# Autodesk Inventor assembly: FTC Drivetrain V2
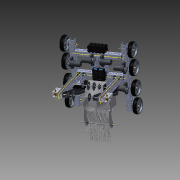
[picture p0: Inventor's stored thumbnail of the model, 180x180]
Saved by Autodesk Inventor 2015 (Build 190159000, 159)
## iProperties
Created: 2014-08-16
Part Number: FTC Drivetrain V2
Document SubType Name: Assembly
Designer: Vinay
Mass: 2195.41 g
Surface Area: 12375.9 cm^2
Volume: 2195.41 cm^3
Density: 1 g/cm^3
Author: Vinay
## Documents named in this file (38)
- C:\Working Folder\FTC Drivetrain V3.iam
- C:\Working Folder\CAD Models\Imported Components\Pitsco Education-739069\Pitsco Education-739069.ipt
- C:\Working Folder\CAD Models\FTC_Tetrix_KOP_Block_Party\Tetrix_Kit_FTC\Imported Components\tetrix_739089_2012\tetrix_739089_2012.ipt
- C:\Working Folder\CAD Models\FTC_Tetrix_KOP_Block_Party\Tetrix_Kit_FTC\Imported Components\tetrix_739083_motor_2012\tetrix_739083_motor_2012.ipt
- C:\Working Folder\CAD Models\Imported Components\Pitsco Education-739091\Pitsco Education-739091.ipt
- C:\Working Folder\CAD Models\Imported Components\Pitsco Education-739069\Pitsco Education-739069_MIR.ipt
- C:\Working Folder\CAD Models\FTC_Tetrix_KOP_Block_Party\Tetrix_Kit_FTC\Imported Components\tetrix_739089_2012\tetrix_739089_2012_MIR.ipt
- C:\Working Folder\CAD Models\FTC_Tetrix_KOP_Block_Party\Tetrix_Kit_FTC\Imported Components\tetrix_739083_motor_2012\tetrix_739083_motor_2012_MIR.ipt
- C:\Working Folder\CAD Models\Imported Components\Pitsco Education-739091\Pitsco Education-739091_MIR.ipt
- C:\Working Folder\CAD Models\FTC_Tetrix_KOP_Block_Party\Tetrix_Kit_FTC\Imported Components\tetrix_739062_2012\tetrix_739062_2012.ipt
- C:\Working Folder\CAD Models\Imported Components\Pitsco Education-739068\Pitsco Education-739068.ipt
- C:\Working Folder\CAD Models\FTC_Tetrix_KOP_Block_Party\Tetrix_Kit_FTC\Imported Components\tetrix_739088_2013\tetrix_739088_2013.ipt
- C:\Working Folder\CAD Models\FTC_Tetrix_KOP_Block_Party\Tetrix_Kit_FTC\Imported Components\tetrix_739079_2012\tetrix_739079_2012.iam
- C:\Working Folder\CAD Models\FTC_Tetrix_KOP_Block_Party\Tetrix_Kit_FTC\Imported Components\tetrix_739172_2012\tetrix_739172_2012.iam
- C:\Working Folder\CAD Models\Imported Components\Pitsco Education-739169\Pitsco Education-739169.ipt
- C:\Working Folder\CAD Models\FTC_Tetrix_KOP_Block_Party\Tetrix_Kit_FTC\Imported Components\tetrix_739165_sprk_25_16t_2013\tetrix_739165_sprk_25_16t_2013.ipt
- C:\Working Folder\CAD Models\FTC_Tetrix_KOP_Block_Party\Tetrix_Kit_FTC\Imported Components\tetrix_739092_2012\tetrix_739092_2012.iam
- C:\Working Folder\CAD Models\FTC_Tetrix_KOP_Block_Party\Tetrix_Kit_FTC\Imported Components\tetrix_739172_collar_2012\tetrix_739172_collar_2012.ipt
- C:\Working Folder\CAD Models\FTC_Tetrix_KOP_Block_Party\Tetrix_Kit_FTC\Imported Components\tetrix_739100_2012\tetrix_739100_2012.ipt
- C:\Working Folder\CAD Models\FTC_Tetrix_KOP_Block_Party\Tetrix_Kit_FTC\Imported Components\tetrix_739055_2012\tetrix_739055_2012.ipt
- C:\Working Folder\CAD Models\Imported Components\Pitsco Education-739066\Pitsco Education-739066.ipt
- C:\Working Folder\CAD Models\FTC_Tetrix_KOP_Block_Party\Tetrix_Kit_FTC\Imported Components\tetrix_739089_2012\tetrix_739089_2012_MIR1.ipt
- C:\Working Folder\CAD Models\FTC_Tetrix_KOP_Block_Party\Tetrix_Kit_FTC\Imported Components\tetrix_739083_motor_2012\tetrix_739083_motor_2012_MIR1.ipt
- C:\Working Folder\CAD Models\FTC_Tetrix_KOP_Block_Party\Tetrix_Kit_FTC\Imported Components\tetrix_739079_2012\tetrix_739079_2012_MIR.iam
- C:\Working Folder\CAD Models\FTC_Tetrix_KOP_Block_Party\Tetrix_Kit_FTC\Imported Components\tetrix_739165_sprk_25_16t_2013\tetrix_739165_sprk_25_16t_2013_MIR.ipt
- C:\Working Folder\CAD Models\Imported Components\Pitsco Education-739066\Pitsco Education-739066_MIR.ipt
- C:\Working Folder\CAD Models\FTC_Tetrix_KOP_Block_Party\Tetrix_Kit_FTC\Imported Components\tetrix_739089_2012\tetrix_739089_2012_MIR1_MIR.ipt
- C:\Working Folder\CAD Models\FTC_Tetrix_KOP_Block_Party\Tetrix_Kit_FTC\Imported Components\tetrix_739083_motor_2012\tetrix_739083_motor_2012_MIR1_MIR.ipt
- C:\Working Folder\CAD Models\FTC_Tetrix_KOP_Block_Party\Tetrix_Kit_FTC\Imported Components\tetrix_739079_2012\tetrix_739079_2012_MIR_MIR.iam
- C:\Working Folder\CAD Models\FTC_Tetrix_KOP_Block_Party\Tetrix_Kit_FTC\Imported Components\tetrix_739165_sprk_25_16t_2013\tetrix_739165_sprk_25_16t_2013_MIR_MIR.ipt
- C:\Working Folder\CAD Models\Long Axle 250mm.ipt
- C:\Working Folder\CAD Models\FTC_Tetrix_KOP_Block_Party\Tetrix_Kit_FTC\Imported Components\tetrix_739169_sprk_25_24t_2013\tetrix_739169_sprk_25_24t_2013.ipt
- C:\Working Folder\CAD Models\FTC_Tetrix_KOP_Block_Party\Tetrix_Kit_FTC\Imported Components\tetrix_739169_2012\tetrix_739169_2012.ipt
- C:\Working Folder\CAD Models\FTC_Tetrix_KOP_Block_Party\Tetrix_Kit_FTC\Imported Components\tetrix_739068_2012\tetrix_739068_2012.ipt
- C:\Working Folder\CAD Models\FTC_Tetrix_KOP_Block_Party\Tetrix_Kit_FTC\Imported Components\tetrix_991444_2012\tetrix_991444_2012.ipt
- C:\Working Folder\CAD Models\FTC_Tetrix_KOP_Block_Party\Tetrix_Kit_FTC\Imported Components\tetrix_739057_2012\tetrix_739057_2012.ipt
- C:\Working Folder\CAD Models\Imported Components\Pitsco Education-739375\Pitsco Education-739375.iam
- C:\Working Folder\CAD Models\GAME ELEMENT FINAL.iam
## Components (151 placed, 37 different names)
1. Pitsco Education-739069:1 — Mate:11, Mate:12, Mate:13, Mate:14, Mate:17, Mate:18, Mate:19, Mate:20, Mate:21, Mate:22, Mate:23, Mate:24, Mate:49, Mate:50, Mate:51, Mate:61, Mate:62, Mate:63, Mate:70, Mate:71, Mate:72, Mate:73, Flush:8, Flush:9, Flush:10, Flush:11, Mate:235, Mate:236, Mate:237, Mate:238, Mate:239, Mate:240, Mate:335, Flush:23
2. tetrix_739089_2012:1 — Mate:7, Flush:2, Mate:235, Mate:236, Mate:237
3. tetrix_739089_2012:2 — Mate:8, Flush:1, Mate:238, Mate:239, Mate:240
4. tetrix_739083_motor_2012:1 — Mate:7, Flush:2, Mate:86, Mate:87
5. tetrix_739083_motor_2012:2 — Mate:8, Flush:1, Mate:88, Mate:89
6. Pitsco Education-739091:1 — Mate:11, Mate:12, Mate:134, Mate:135
7. Pitsco Education-739091:3 — Mate:13, Mate:14, Mate:85, Mate:94
8. Pitsco Education-739091:4 — Mate:72, Mate:73, Mate:82, Mate:100
9. Pitsco Education-739091:5 — Mate:23, Mate:24, Mate:146, Mate:147
10. Pitsco Education-739091:6 — Mate:70, Mate:71, Mate:84, Mate:96
11. Pitsco Education-739091:7 — Mate:21, Mate:22, Mate:142, Mate:143
12. Pitsco Education-739091:10 — Mate:19, Mate:20, Mate:136, Mate:137
13. Pitsco Education-739091:11 — Mate:17, Mate:18, Mate:83, Mate:98
14. Pitsco Education-739069_MIR:1 — Mate:33, Mate:34, Mate:35, Mate:36, Mate:39, Mate:40, Mate:43, Mate:44, Mate:45, Mate:46, Mate:47, Mate:48, Mate:58, Mate:59, Mate:60, Mate:74, Mate:75, Mate:76, Mate:77, Flush:5, Flush:6, Mate:150, Flush:7, Mate:241, Mate:242, Mate:243, Mate:244, Mate:245, Mate:246
15. tetrix_739089_2012_MIR:1 — Flush:3, Mate:31, Mate:241, Mate:242, Mate:243
16. tetrix_739089_2012_MIR:2 — Flush:4, Mate:32, Mate:244, Mate:245, Mate:246
17. tetrix_739083_motor_2012_MIR:1 — Flush:3, Mate:31, Mate:90, Mate:91
18. tetrix_739083_motor_2012_MIR:2 — Flush:4, Mate:32, Mate:92, Mate:93
19. Pitsco Education-739091_MIR:1 — Mate:33, Mate:34, Mate:140, Mate:141
20. Pitsco Education-739091_MIR:2 — Mate:35, Mate:36, Mate:81, Mate:108
21. Pitsco Education-739091_MIR:3 — Mate:76, Mate:77, Mate:78, Mate:106
22. Pitsco Education-739091_MIR:4 — Mate:39, Mate:40, Mate:148, Mate:149
23. Pitsco Education-739091_MIR:5 — Mate:74, Mate:75, Mate:80, Mate:102
24. Pitsco Education-739091_MIR:6 — Mate:43, Mate:44, Mate:144, Mate:145
25. Pitsco Education-739091_MIR:7 — Mate:45, Mate:46, Mate:138, Mate:139
26. Pitsco Education-739091_MIR:8 — Mate:47, Mate:48, Mate:79, Mate:104
27. tetrix_739062_2012:2 — Mate:49, Mate:50, Mate:51, Mate:52, Mate:53, Mate:54
28. Pitsco Education-739068:1 — Mate:52, Mate:53, Mate:54, Mate:55, Mate:56, Mate:57, Mate:276, Mate:277, Flush:14, Flush:16, Mate:286, Mate:287, Mate:336
29. tetrix_739062_2012:5 — Mate:55, Mate:56, Mate:57, Mate:58, Mate:59, Mate:60
30. tetrix_739062_2012:6 — Mate:61, Mate:62, Mate:63, Mate:64, Mate:65, Mate:66, Mate:216
31. tetrix_739062_2012:7 — Mate:67, Mate:68, Mate:69
32. Pitsco Education-739068:2 — Mate:64, Mate:65, Mate:66, Mate:67, Mate:68, Mate:69, Mate:215, Mate:217, Mate:220, Mate:221, Mate:222, Mate:225, Mate:226, Mate:227, Mate:229, Mate:230, Mate:278, Mate:288, Mate:328, Mate:329
33. tetrix_739088_2013:1 — Mate:81, Mate:109, Flush:6, Mate:174, Mate:182, Mate:190
34. tetrix_739088_2013:2 — Mate:80, Mate:103, Flush:7, Mate:172, Mate:180, Mate:188, Mate:196
35. tetrix_739088_2013:3 — Mate:79, Mate:105, Mate:150, Mate:170, Mate:178, Mate:186, Mate:194
36. tetrix_739088_2013:4 — Mate:78, Mate:107, Flush:5, Mate:167, Mate:176, Mate:184
37. tetrix_739088_2013:5 — Mate:85, Mate:95, Flush:11, Mate:158, Mate:164, Mate:200
38. tetrix_739088_2013:6 — Mate:84, Mate:97, Flush:10, Mate:154, Mate:166, Mate:202
39. tetrix_739088_2013:7 — Mate:83, Mate:99, Flush:9, Mate:155, Mate:162, Mate:204
40. tetrix_739088_2013:8 — Mate:82, Mate:101, Flush:8, Mate:152, Mate:160, Mate:206
41. tetrix_739079_2012:1 [sub-assembly] — Mate:88, Mate:89, Mate:112, Mate:113
42. tetrix_739079_2012:2 [sub-assembly] — Mate:86, Mate:87, Mate:116, Mate:117
43. tetrix_739079_2012:3 [sub-assembly] — Mate:92, Mate:93, Mate:122, Mate:123
44. tetrix_739079_2012:4 [sub-assembly] — Mate:90, Mate:91, Mate:132, Mate:133
45. tetrix_739172_2012:1 [sub-assembly] — Mate:94, Mate:95, Mate:110, Mate:111
46. tetrix_739172_2012:2 [sub-assembly] — Mate:100, Mate:101, Mate:120, Mate:121
47. tetrix_739172_2012:3 [sub-assembly] — Mate:98, Mate:99, Mate:118, Mate:119
48. tetrix_739172_2012:4 [sub-assembly] — Mate:96, Mate:97, Mate:114, Mate:115
49. tetrix_739172_2012:6 [sub-assembly] — Mate:104, Mate:105, Mate:126, Mate:127
50. tetrix_739172_2012:7 [sub-assembly] — Mate:106, Mate:107, Mate:124, Mate:125
51. tetrix_739172_2012:8 [sub-assembly] — Mate:108, Mate:109, Mate:130, Mate:131
52. Pitsco Education-739169:1 — Mate:110, Mate:111, Mate:157
53. Pitsco Education-739169:2 — Mate:114, Mate:115, Mate:153
54. Pitsco Education-739169:3 — Mate:118, Mate:119, Mate:156
55. Pitsco Education-739169:4 — Mate:120, Mate:121, Mate:151
56. tetrix_739165_sprk_25_16t_2013:1 — Mate:122, Mate:123
57. tetrix_739165_sprk_25_16t_2013:2 — Mate:112, Mate:113
58. tetrix_739165_sprk_25_16t_2013:3 — Mate:116, Mate:117
59. Pitsco Education-739169:5 — Mate:124, Mate:125, Mate:168
60. Pitsco Education-739169:6 — Mate:126, Mate:127, Mate:169
61. Pitsco Education-739169:7 — Mate:130, Mate:131, Mate:173
62. Pitsco Education-739169:8 — Mate:128, Mate:129, Mate:171
63. tetrix_739165_sprk_25_16t_2013:4 — Mate:132, Mate:133
64. tetrix_739092_2012:1 [sub-assembly] — Mate:138, Mate:139
65. tetrix_739092_2012:2 [sub-assembly] — Mate:142, Mate:143
66. tetrix_739172_2012:5 [sub-assembly] — Mate:102, Mate:103, Mate:128, Mate:129
67. tetrix_739092_2012:3 [sub-assembly] — Mate:140, Mate:141
68. tetrix_739092_2012:4 [sub-assembly] — Mate:146, Mate:147
69. tetrix_739092_2012:5 [sub-assembly] — Mate:136, Mate:137
70. tetrix_739092_2012:6 [sub-assembly] — Mate:144, Mate:145
71. tetrix_739092_2012:7 [sub-assembly] — Mate:148, Mate:149
72. tetrix_739092_2012:8 [sub-assembly] — Mate:134, Mate:135
73. tetrix_739172_collar_2012:1 — Mate:163, Mate:164, Mate:199
74. tetrix_739172_collar_2012:2 — Mate:161, Mate:162, Mate:203
75. tetrix_739172_collar_2012:3 — Mate:159, Mate:160, Mate:205
76. tetrix_739172_collar_2012:4 — Mate:165, Mate:166, Mate:201
77. tetrix_739100_2012:1 — Mate:155, Mate:156, Mate:161
78. tetrix_739100_2012:2 — Mate:151, Mate:152, Mate:159
79. tetrix_739100_2012:3 — Mate:153, Mate:154, Mate:165
80. tetrix_739100_2012:4 — Mate:157, Mate:158, Mate:163
81. tetrix_739100_2012:5 — Mate:167, Mate:168, Mate:175
82. tetrix_739100_2012:6 — Mate:173, Mate:174, Mate:181
83. tetrix_739100_2012:7 — Mate:171, Mate:172, Mate:179
84. tetrix_739100_2012:8 — Mate:169, Mate:170, Mate:177
85. tetrix_739172_2012:9 [sub-assembly] — Mate:175, Mate:176, Mate:183
86. tetrix_739172_2012:10 [sub-assembly] — Mate:179, Mate:180, Mate:187
87. tetrix_739172_2012:11 [sub-assembly] — Mate:177, Mate:178, Mate:185
88. tetrix_739172_2012:12 [sub-assembly] — Mate:181, Mate:182, Mate:189
89. Pitsco Education-739091:12 — Mate:183, Mate:184, Mate:191, Mate:192
90. Pitsco Education-739091:13 — Mate:185, Mate:186, Mate:193
91. Pitsco Education-739091:14 — Mate:189, Mate:190, Mate:197, Mate:198
92. Pitsco Education-739091:15 — Mate:187, Mate:188, Mate:195
93. tetrix_739055_2012:1 — Mate:191, Mate:192
94. tetrix_739055_2012:2 — Mate:193, Mate:194
95. tetrix_739055_2012:3 — Mate:197, Mate:198
96. tetrix_739055_2012:4 — Mate:195, Mate:196
97. Pitsco Education-739091:16 — Mate:205, Mate:206, Mate:207, Mate:208
98. Pitsco Education-739091:17 — Mate:203, Mate:204, Mate:209, Mate:210
99. Pitsco Education-739091:18 — Mate:201, Mate:202, Mate:211, Mate:212
100. Pitsco Education-739091:19 — Mate:199, Mate:200, Mate:213, Mate:214
101. tetrix_739055_2012:5 — Mate:207, Mate:208
102. tetrix_739055_2012:6 — Mate:209, Mate:210
103. tetrix_739055_2012:7 — Mate:211, Mate:212
104. tetrix_739055_2012:8 — Mate:213, Mate:214
105. Pitsco Education-739068:3 — Mate:223, Mate:224, Mate:234, Mate:249, Mate:263, Mate:290, Mate:293, Mate:334, Mate:338, Flush:24, Mate:339, Mate:343
106. Pitsco Education-739068:4 — Mate:218, Mate:219, Mate:251, Mate:257, Mate:268, Mate:291, Mate:294, Mate:295, Mate:297, Mate:325, Mate:331, Mate:332, Mate:340, Flush:25, Mate:341
107. Pitsco Education-739066:1 — Mate:228, Mate:231, Mate:268, Mate:330
108. Pitsco Education-739066:2 — Mate:232, Mate:233, Mate:234, Mate:333
109. tetrix_739062_2012:8 — Mate:215, Mate:216, Mate:217, Mate:218, Mate:219
110. tetrix_739062_2012:9 — Mate:220, Mate:221, Mate:222, Mate:223, Mate:224
111. tetrix_739062_2012:10 — Mate:225, Mate:226, Mate:227, Mate:228, Mate:231
112. tetrix_739062_2012:11 — Mate:229, Mate:230, Mate:232, Mate:233
113. Pitsco Education-739091:20 — Mate:249, Mate:293
114. Pitsco Education-739091:21 — Mate:251, Mate:294, Mate:296
115. Pitsco Education-739091:24 — Mate:257, Mate:291
116. Pitsco Education-739091:25 — Mate:263, Mate:290, Mate:292
117. Pitsco Education-739066:3 — Flush:14, Mate:278, Mate:279
118. tetrix_739089_2012_MIR1:1 — Flush:13, Mate:271, Mate:276, Mate:277, Mate:279
119. tetrix_739083_motor_2012_MIR1:1 — Flush:13, Mate:271, Mate:272, Mate:273
120. tetrix_739079_2012_MIR:1 [sub-assembly] — Mate:272, Mate:273, Mate:274, Mate:275
121. tetrix_739165_sprk_25_16t_2013_MIR:1 — Mate:274, Mate:275, Flush:17
122. Pitsco Education-739066_MIR:1 — Mate:280, Flush:16, Mate:288
123. tetrix_739089_2012_MIR1_MIR:1 — Mate:280, Mate:281, Flush:15, Mate:286, Mate:287
124. tetrix_739083_motor_2012_MIR1_MIR:1 — Mate:281, Flush:15, Mate:282, Mate:283
125. tetrix_739079_2012_MIR_MIR:1 [sub-assembly] — Mate:282, Mate:283, Mate:284, Mate:285
126. tetrix_739165_sprk_25_16t_2013_MIR_MIR:1 — Mate:284, Mate:285, Flush:18
127. Long Axle 250mm:1 — Mate:295, Mate:296, Mate:298, Mate:299, Mate:300, Mate:301
128. Long Axle 250mm:2 — Mate:292, Mate:297, Mate:305, Mate:318, Mate:320, Mate:323, Mate:324, Mate:337
129. tetrix_739169_sprk_25_24t_2013:1 — Mate:298, Flush:17, Mate:303, Mate:314, Mate:315
130. tetrix_739169_sprk_25_24t_2013:2 — Mate:299, Flush:18, Mate:302, Mate:312, Mate:313
131. tetrix_739165_sprk_25_16t_2013:5 — Mate:300, Mate:303, Flush:19, Mate:316, Mate:317
132. tetrix_739165_sprk_25_16t_2013:7 — Mate:301, Mate:302, Flush:20, Mate:310, Mate:311
133. tetrix_739169_2012:1 — Flush:20, Mate:306, Mate:307, Mate:337
134. tetrix_739169_2012:2 — Mate:305, Flush:19, Mate:308, Mate:309
135. tetrix_739172_collar_2012:5 — Mate:310, Mate:311
136. tetrix_739172_collar_2012:6 — Mate:312, Mate:313
137. tetrix_739172_collar_2012:7 — Mate:314, Mate:315
138. tetrix_739172_collar_2012:8 — Mate:316, Mate:317
139. tetrix_739172_collar_2012:9 — Mate:308, Mate:309
140. tetrix_739172_collar_2012:10 — Mate:306, Mate:307
141. tetrix_739068_2012:2 — Mate:320, Mate:321, Mate:343
142. tetrix_739172_collar_2012:12 — Mate:318, Mate:321
143. tetrix_739068_2012:3 — Mate:323, Mate:325, Mate:326, Mate:344
144. tetrix_739172_collar_2012:13 — Mate:324, Mate:326
145. tetrix_991444_2012:3 — Mate:328, Mate:329
146. tetrix_991444_2012:4 — Mate:333, Mate:334, Flush:22
147. tetrix_991444_2012:5 — Mate:330, Mate:331, Mate:332, Flush:22
148. tetrix_739057_2012:1 — Mate:335, Flush:23, Mate:336
149. Pitsco Education-739375:1 [sub-assembly] — Mate:340, Flush:25, Mate:341
150. Pitsco Education-739375:2 [sub-assembly] — Mate:338, Flush:24, Mate:339
151. GAME ELEMENT FINAL:1 [sub-assembly] — Mate:344
## Relationships (322: Mate 299, Flush 23)
- Mate:7: tetrix_739089_2012:1 ↔ tetrix_739083_motor_2012:1
- Mate:8: tetrix_739089_2012:2 ↔ tetrix_739083_motor_2012:2
- Flush:1: tetrix_739089_2012:2 ↔ tetrix_739083_motor_2012:2
- Flush:2: tetrix_739089_2012:1 ↔ tetrix_739083_motor_2012:1
- Mate:11: Pitsco Education-739069:1 ↔ Pitsco Education-739091:1
- Mate:12: Pitsco Education-739069:1 ↔ Pitsco Education-739091:1
- Mate:13: Pitsco Education-739069:1 ↔ Pitsco Education-739091:3
- Mate:14: Pitsco Education-739069:1 ↔ Pitsco Education-739091:3
- Mate:17: Pitsco Education-739069:1 ↔ Pitsco Education-739091:11
- Mate:18: Pitsco Education-739069:1 ↔ Pitsco Education-739091:11
- Mate:19: Pitsco Education-739069:1 ↔ Pitsco Education-739091:10
- Mate:20: Pitsco Education-739069:1 ↔ Pitsco Education-739091:10
- Mate:21: Pitsco Education-739069:1 ↔ Pitsco Education-739091:7
- Mate:22: Pitsco Education-739069:1 ↔ Pitsco Education-739091:7
- Mate:23: Pitsco Education-739069:1 ↔ Pitsco Education-739091:5
- Mate:24: Pitsco Education-739069:1 ↔ Pitsco Education-739091:5
- Flush:3: tetrix_739089_2012_MIR:1 ↔ tetrix_739083_motor_2012_MIR:1
- Mate:31: tetrix_739089_2012_MIR:1 ↔ tetrix_739083_motor_2012_MIR:1
- Flush:4: tetrix_739089_2012_MIR:2 ↔ tetrix_739083_motor_2012_MIR:2
- Mate:32: tetrix_739089_2012_MIR:2 ↔ tetrix_739083_motor_2012_MIR:2
- Mate:33: Pitsco Education-739069_MIR:1 ↔ Pitsco Education-739091_MIR:1
- Mate:34: Pitsco Education-739069_MIR:1 ↔ Pitsco Education-739091_MIR:1
- Mate:35: Pitsco Education-739069_MIR:1 ↔ Pitsco Education-739091_MIR:2
- Mate:36: Pitsco Education-739069_MIR:1 ↔ Pitsco Education-739091_MIR:2
- Mate:39: Pitsco Education-739069_MIR:1 ↔ Pitsco Education-739091_MIR:4
- Mate:40: Pitsco Education-739069_MIR:1 ↔ Pitsco Education-739091_MIR:4
- Mate:43: Pitsco Education-739069_MIR:1 ↔ Pitsco Education-739091_MIR:6
- Mate:44: Pitsco Education-739069_MIR:1 ↔ Pitsco Education-739091_MIR:6
- Mate:45: Pitsco Education-739069_MIR:1 ↔ Pitsco Education-739091_MIR:7
- Mate:46: Pitsco Education-739069_MIR:1 ↔ Pitsco Education-739091_MIR:7
- Mate:47: Pitsco Education-739069_MIR:1 ↔ Pitsco Education-739091_MIR:8
- Mate:48: Pitsco Education-739069_MIR:1 ↔ Pitsco Education-739091_MIR:8
- Mate:49: Pitsco Education-739069:1 ↔ tetrix_739062_2012:2
- Mate:50: Pitsco Education-739069:1 ↔ tetrix_739062_2012:2
- Mate:51: Pitsco Education-739069:1 ↔ tetrix_739062_2012:2
- Mate:52: tetrix_739062_2012:2 ↔ Pitsco Education-739068:1
- Mate:53: tetrix_739062_2012:2 ↔ Pitsco Education-739068:1
- Mate:54: tetrix_739062_2012:2 ↔ Pitsco Education-739068:1
- Mate:55: Pitsco Education-739068:1 ↔ tetrix_739062_2012:5
- Mate:56: Pitsco Education-739068:1 ↔ tetrix_739062_2012:5
- Mate:57: Pitsco Education-739068:1 ↔ tetrix_739062_2012:5
- Mate:58: Pitsco Education-739069_MIR:1 ↔ tetrix_739062_2012:5
- Mate:59: Pitsco Education-739069_MIR:1 ↔ tetrix_739062_2012:5
- Mate:60: Pitsco Education-739069_MIR:1 ↔ tetrix_739062_2012:5
- Mate:61: Pitsco Education-739069:1 ↔ tetrix_739062_2012:6
- Mate:62: Pitsco Education-739069:1 ↔ tetrix_739062_2012:6
- Mate:63: Pitsco Education-739069:1 ↔ tetrix_739062_2012:6
- Mate:64: tetrix_739062_2012:6 ↔ Pitsco Education-739068:2
- Mate:65: tetrix_739062_2012:6 ↔ Pitsco Education-739068:2
- Mate:66: tetrix_739062_2012:6 ↔ Pitsco Education-739068:2
- Mate:67: tetrix_739062_2012:7 ↔ Pitsco Education-739068:2
- Mate:68: tetrix_739062_2012:7 ↔ Pitsco Education-739068:2
- Mate:69: tetrix_739062_2012:7 ↔ Pitsco Education-739068:2
- Mate:70: Pitsco Education-739069:1 ↔ Pitsco Education-739091:6
- Mate:71: Pitsco Education-739069:1 ↔ Pitsco Education-739091:6
- Mate:72: Pitsco Education-739069:1 ↔ Pitsco Education-739091:4
- Mate:73: Pitsco Education-739069:1 ↔ Pitsco Education-739091:4
- Mate:74: Pitsco Education-739069_MIR:1 ↔ Pitsco Education-739091_MIR:5
- Mate:75: Pitsco Education-739069_MIR:1 ↔ Pitsco Education-739091_MIR:5
- Mate:76: Pitsco Education-739069_MIR:1 ↔ Pitsco Education-739091_MIR:3
- Mate:77: Pitsco Education-739069_MIR:1 ↔ Pitsco Education-739091_MIR:3
- Mate:78: Pitsco Education-739091_MIR:3 ↔ tetrix_739088_2013:4
- Mate:79: Pitsco Education-739091_MIR:8 ↔ tetrix_739088_2013:3
- Mate:80: Pitsco Education-739091_MIR:5 ↔ tetrix_739088_2013:2
- Mate:81: Pitsco Education-739091_MIR:2 ↔ tetrix_739088_2013:1
- Mate:82: Pitsco Education-739091:4 ↔ tetrix_739088_2013:8
- Mate:83: Pitsco Education-739091:11 ↔ tetrix_739088_2013:7
- Mate:84: Pitsco Education-739091:6 ↔ tetrix_739088_2013:6
- Mate:85: Pitsco Education-739091:3 ↔ tetrix_739088_2013:5
- Mate:86: tetrix_739083_motor_2012:1 ↔ tetrix_739079_2012:2
- Mate:87: tetrix_739083_motor_2012:1 ↔ tetrix_739079_2012:2
- Mate:88: tetrix_739083_motor_2012:2 ↔ tetrix_739079_2012:1
- Mate:89: tetrix_739083_motor_2012:2 ↔ tetrix_739079_2012:1
- Mate:90: tetrix_739083_motor_2012_MIR:1 ↔ tetrix_739079_2012:4
- Mate:91: tetrix_739083_motor_2012_MIR:1 ↔ tetrix_739079_2012:4
- Mate:92: tetrix_739083_motor_2012_MIR:2 ↔ tetrix_739079_2012:3
- Mate:93: tetrix_739083_motor_2012_MIR:2 ↔ tetrix_739079_2012:3
- Mate:94: Pitsco Education-739091:3 ↔ tetrix_739172_2012:1
- Mate:95: tetrix_739088_2013:5 ↔ tetrix_739172_2012:1
- Mate:96: Pitsco Education-739091:6 ↔ tetrix_739172_2012:4
- Mate:97: tetrix_739088_2013:6 ↔ tetrix_739172_2012:4
- Mate:98: Pitsco Education-739091:11 ↔ tetrix_739172_2012:3
- Mate:99: tetrix_739088_2013:7 ↔ tetrix_739172_2012:3
- Mate:100: Pitsco Education-739091:4 ↔ tetrix_739172_2012:2
- Mate:101: tetrix_739088_2013:8 ↔ tetrix_739172_2012:2
- Mate:102: Pitsco Education-739091_MIR:5 ↔ tetrix_739172_2012:5
- Mate:103: tetrix_739088_2013:2 ↔ tetrix_739172_2012:5
- Mate:104: Pitsco Education-739091_MIR:8 ↔ tetrix_739172_2012:6
- Mate:105: tetrix_739088_2013:3 ↔ tetrix_739172_2012:6
- Mate:106: Pitsco Education-739091_MIR:3 ↔ tetrix_739172_2012:7
- Mate:107: tetrix_739088_2013:4 ↔ tetrix_739172_2012:7
- Mate:108: Pitsco Education-739091_MIR:2 ↔ tetrix_739172_2012:8
- Mate:109: tetrix_739088_2013:1 ↔ tetrix_739172_2012:8
- Mate:110: tetrix_739172_2012:1 ↔ Pitsco Education-739169:1
- Mate:111: tetrix_739172_2012:1 ↔ Pitsco Education-739169:1
- Mate:112: tetrix_739079_2012:1 ↔ tetrix_739165_sprk_25_16t_2013:2
- Mate:113: tetrix_739079_2012:1 ↔ tetrix_739165_sprk_25_16t_2013:2
- Mate:114: tetrix_739172_2012:4 ↔ Pitsco Education-739169:2
- Mate:115: tetrix_739172_2012:4 ↔ Pitsco Education-739169:2
- Mate:116: tetrix_739079_2012:2 ↔ tetrix_739165_sprk_25_16t_2013:3
- Mate:117: tetrix_739079_2012:2 ↔ tetrix_739165_sprk_25_16t_2013:3
- Mate:118: tetrix_739172_2012:3 ↔ Pitsco Education-739169:3
- Mate:119: tetrix_739172_2012:3 ↔ Pitsco Education-739169:3
- Mate:120: tetrix_739172_2012:2 ↔ Pitsco Education-739169:4
- Mate:121: tetrix_739172_2012:2 ↔ Pitsco Education-739169:4
- Mate:122: tetrix_739079_2012:3 ↔ tetrix_739165_sprk_25_16t_2013:1
- Mate:123: tetrix_739079_2012:3 ↔ tetrix_739165_sprk_25_16t_2013:1
- Mate:124: tetrix_739172_2012:7 ↔ Pitsco Education-739169:5
- Mate:125: tetrix_739172_2012:7 ↔ Pitsco Education-739169:5
- Mate:126: tetrix_739172_2012:6 ↔ Pitsco Education-739169:6
- Mate:127: tetrix_739172_2012:6 ↔ Pitsco Education-739169:6
- Mate:128: Pitsco Education-739169:8 ↔ tetrix_739172_2012:5
- Mate:129: Pitsco Education-739169:8 ↔ tetrix_739172_2012:5
- Mate:130: tetrix_739172_2012:8 ↔ Pitsco Education-739169:7
- Mate:131: tetrix_739172_2012:8 ↔ Pitsco Education-739169:7
- Mate:132: tetrix_739079_2012:4 ↔ tetrix_739165_sprk_25_16t_2013:4
- Mate:133: tetrix_739079_2012:4 ↔ tetrix_739165_sprk_25_16t_2013:4
- Mate:134: Pitsco Education-739091:1 ↔ tetrix_739092_2012:8
- Mate:135: Pitsco Education-739091:1 ↔ tetrix_739092_2012:8
- Mate:136: Pitsco Education-739091:10 ↔ tetrix_739092_2012:5
- Mate:137: Pitsco Education-739091:10 ↔ tetrix_739092_2012:5
- Mate:138: Pitsco Education-739091_MIR:7 ↔ tetrix_739092_2012:1
- Mate:139: Pitsco Education-739091_MIR:7 ↔ tetrix_739092_2012:1
- Mate:140: Pitsco Education-739091_MIR:1 ↔ tetrix_739092_2012:3
- Mate:141: Pitsco Education-739091_MIR:1 ↔ tetrix_739092_2012:3
- Mate:142: Pitsco Education-739091:7 ↔ tetrix_739092_2012:2
- Mate:143: Pitsco Education-739091:7 ↔ tetrix_739092_2012:2
- Mate:144: Pitsco Education-739091_MIR:6 ↔ tetrix_739092_2012:6
- Mate:145: Pitsco Education-739091_MIR:6 ↔ tetrix_739092_2012:6
- Mate:146: Pitsco Education-739091:5 ↔ tetrix_739092_2012:4
- Mate:147: Pitsco Education-739091:5 ↔ tetrix_739092_2012:4
- Mate:148: Pitsco Education-739091_MIR:4 ↔ tetrix_739092_2012:7
- Mate:149: Pitsco Education-739091_MIR:4 ↔ tetrix_739092_2012:7
- Flush:5 (-12.7 mm): Pitsco Education-739069_MIR:1 ↔ tetrix_739088_2013:4
- Flush:6 (12.7 mm): Pitsco Education-739069_MIR:1 ↔ tetrix_739088_2013:1
- Mate:150 (12.7 mm): Pitsco Education-739069_MIR:1 ↔ tetrix_739088_2013:3
- Flush:7 (-12.7 mm): Pitsco Education-739069_MIR:1 ↔ tetrix_739088_2013:2
- Flush:8 (-12.7 mm): Pitsco Education-739069:1 ↔ tetrix_739088_2013:8
- Flush:9 (-12.7 mm): Pitsco Education-739069:1 ↔ tetrix_739088_2013:7
- Flush:10 (-12.7 mm): Pitsco Education-739069:1 ↔ tetrix_739088_2013:6
- Flush:11 (-12.7 mm): Pitsco Education-739069:1 ↔ tetrix_739088_2013:5
- Mate:151: Pitsco Education-739169:4 ↔ tetrix_739100_2012:2
- Mate:152: tetrix_739088_2013:8 ↔ tetrix_739100_2012:2
- Mate:153: Pitsco Education-739169:2 ↔ tetrix_739100_2012:3
- Mate:154: tetrix_739088_2013:6 ↔ tetrix_739100_2012:3
- Mate:155: tetrix_739088_2013:7 ↔ tetrix_739100_2012:1
- Mate:156: Pitsco Education-739169:3 ↔ tetrix_739100_2012:1
- Mate:157: Pitsco Education-739169:1 ↔ tetrix_739100_2012:4
- Mate:158: tetrix_739088_2013:5 ↔ tetrix_739100_2012:4
- Mate:159: tetrix_739172_collar_2012:3 ↔ tetrix_739100_2012:2
- Mate:160: tetrix_739088_2013:8 ↔ tetrix_739172_collar_2012:3
- Mate:161: tetrix_739172_collar_2012:2 ↔ tetrix_739100_2012:1
- Mate:162: tetrix_739088_2013:7 ↔ tetrix_739172_collar_2012:2
- Mate:163: tetrix_739172_collar_2012:1 ↔ tetrix_739100_2012:4
- Mate:164: tetrix_739088_2013:5 ↔ tetrix_739172_collar_2012:1
- Mate:165: tetrix_739172_collar_2012:4 ↔ tetrix_739100_2012:3
- Mate:166: tetrix_739088_2013:6 ↔ tetrix_739172_collar_2012:4
- Mate:167: tetrix_739088_2013:4 ↔ tetrix_739100_2012:5
- Mate:168: Pitsco Education-739169:5 ↔ tetrix_739100_2012:5
- Mate:169: Pitsco Education-739169:6 ↔ tetrix_739100_2012:8
- Mate:170: tetrix_739088_2013:3 ↔ tetrix_739100_2012:8
- Mate:171: Pitsco Education-739169:8 ↔ tetrix_739100_2012:7
- Mate:172: tetrix_739088_2013:2 ↔ tetrix_739100_2012:7
- Mate:173: Pitsco Education-739169:7 ↔ tetrix_739100_2012:6
- Mate:174: tetrix_739088_2013:1 ↔ tetrix_739100_2012:6
- Mate:175: tetrix_739100_2012:5 ↔ tetrix_739172_2012:9
- Mate:176: tetrix_739088_2013:4 ↔ tetrix_739172_2012:9
- Mate:177: tetrix_739100_2012:8 ↔ tetrix_739172_2012:11
- Mate:178: tetrix_739088_2013:3 ↔ tetrix_739172_2012:11
- Mate:179: tetrix_739100_2012:7 ↔ tetrix_739172_2012:10
- Mate:180: tetrix_739088_2013:2 ↔ tetrix_739172_2012:10
- Mate:181: tetrix_739100_2012:6 ↔ tetrix_739172_2012:12
- Mate:182: tetrix_739088_2013:1 ↔ tetrix_739172_2012:12
- Mate:183: tetrix_739172_2012:9 ↔ Pitsco Education-739091:12
- Mate:184: tetrix_739088_2013:4 ↔ Pitsco Education-739091:12
- Mate:185: tetrix_739172_2012:11 ↔ Pitsco Education-739091:13
- Mate:186: tetrix_739088_2013:3 ↔ Pitsco Education-739091:13
- Mate:187: tetrix_739172_2012:10 ↔ Pitsco Education-739091:15
- Mate:188: tetrix_739088_2013:2 ↔ Pitsco Education-739091:15
- Mate:189: tetrix_739172_2012:12 ↔ Pitsco Education-739091:14
- Mate:190: tetrix_739088_2013:1 ↔ Pitsco Education-739091:14
- Mate:191: Pitsco Education-739091:12 ↔ tetrix_739055_2012:1
- Mate:192: Pitsco Education-739091:12 ↔ tetrix_739055_2012:1
- Mate:193: Pitsco Education-739091:13 ↔ tetrix_739055_2012:2
- Mate:194: tetrix_739088_2013:3 ↔ tetrix_739055_2012:2
- Mate:195: Pitsco Education-739091:15 ↔ tetrix_739055_2012:4
- Mate:196: tetrix_739088_2013:2 ↔ tetrix_739055_2012:4
- Mate:197: Pitsco Education-739091:14 ↔ tetrix_739055_2012:3
- Mate:198: Pitsco Education-739091:14 ↔ tetrix_739055_2012:3
- Mate:199: tetrix_739172_collar_2012:1 ↔ Pitsco Education-739091:19
- Mate:200: tetrix_739088_2013:5 ↔ Pitsco Education-739091:19
- Mate:201: tetrix_739172_collar_2012:4 ↔ Pitsco Education-739091:18
- Mate:202: tetrix_739088_2013:6 ↔ Pitsco Education-739091:18
- Mate:203: tetrix_739172_collar_2012:2 ↔ Pitsco Education-739091:17
- Mate:204: tetrix_739088_2013:7 ↔ Pitsco Education-739091:17
- Mate:205: tetrix_739172_collar_2012:3 ↔ Pitsco Education-739091:16
- Mate:206: tetrix_739088_2013:8 ↔ Pitsco Education-739091:16
- Mate:207: Pitsco Education-739091:16 ↔ tetrix_739055_2012:5
- Mate:208: Pitsco Education-739091:16 ↔ tetrix_739055_2012:5
- Mate:209: Pitsco Education-739091:17 ↔ tetrix_739055_2012:6
- Mate:210: Pitsco Education-739091:17 ↔ tetrix_739055_2012:6
- Mate:211: Pitsco Education-739091:18 ↔ tetrix_739055_2012:7
- Mate:212: Pitsco Education-739091:18 ↔ tetrix_739055_2012:7
- Mate:213: Pitsco Education-739091:19 ↔ tetrix_739055_2012:8
- Mate:214: Pitsco Education-739091:19 ↔ tetrix_739055_2012:8
- Mate:215: Pitsco Education-739068:2 ↔ tetrix_739062_2012:8
- Mate:216: tetrix_739062_2012:6 ↔ tetrix_739062_2012:8
- Mate:217: Pitsco Education-739068:2 ↔ tetrix_739062_2012:8
- Mate:218: Pitsco Education-739068:4 ↔ tetrix_739062_2012:8
- Mate:219: Pitsco Education-739068:4 ↔ tetrix_739062_2012:8
- Mate:220: Pitsco Education-739068:2 ↔ tetrix_739062_2012:9
- Mate:221: Pitsco Education-739068:2 ↔ tetrix_739062_2012:9
- Mate:222: Pitsco Education-739068:2 ↔ tetrix_739062_2012:9
- Mate:223: Pitsco Education-739068:3 ↔ tetrix_739062_2012:9
- Mate:224: Pitsco Education-739068:3 ↔ tetrix_739062_2012:9
- Mate:225: Pitsco Education-739068:2 ↔ tetrix_739062_2012:10
- Mate:226: Pitsco Education-739068:2 ↔ tetrix_739062_2012:10
- Mate:227: Pitsco Education-739068:2 ↔ tetrix_739062_2012:10
- Mate:228: Pitsco Education-739066:1 ↔ tetrix_739062_2012:10
- Mate:229: Pitsco Education-739068:2 ↔ tetrix_739062_2012:11
- Mate:230: Pitsco Education-739068:2 ↔ tetrix_739062_2012:11
- Mate:231: Pitsco Education-739066:1 ↔ tetrix_739062_2012:10
- Mate:232: Pitsco Education-739066:2 ↔ tetrix_739062_2012:11
- Mate:233: Pitsco Education-739066:2 ↔ tetrix_739062_2012:11
- Mate:234: Pitsco Education-739068:3 ↔ Pitsco Education-739066:2
- Mate:235: Pitsco Education-739069:1 ↔ tetrix_739089_2012:1
- Mate:236: Pitsco Education-739069:1 ↔ tetrix_739089_2012:1
- Mate:237: Pitsco Education-739069:1 ↔ tetrix_739089_2012:1
- Mate:238: Pitsco Education-739069:1 ↔ tetrix_739089_2012:2
- Mate:239: Pitsco Education-739069:1 ↔ tetrix_739089_2012:2
- Mate:240: Pitsco Education-739069:1 ↔ tetrix_739089_2012:2
- Mate:241: Pitsco Education-739069_MIR:1 ↔ tetrix_739089_2012_MIR:1
- Mate:242: Pitsco Education-739069_MIR:1 ↔ tetrix_739089_2012_MIR:1
- Mate:243: Pitsco Education-739069_MIR:1 ↔ tetrix_739089_2012_MIR:1
- Mate:244: Pitsco Education-739069_MIR:1 ↔ tetrix_739089_2012_MIR:2
- Mate:245: Pitsco Education-739069_MIR:1 ↔ tetrix_739089_2012_MIR:2
- Mate:246: Pitsco Education-739069_MIR:1 ↔ tetrix_739089_2012_MIR:2
- Mate:249: Pitsco Education-739068:3 ↔ Pitsco Education-739091:20
- Mate:251: Pitsco Education-739068:4 ↔ Pitsco Education-739091:21
- Mate:257: Pitsco Education-739068:4 ↔ Pitsco Education-739091:24
- Mate:263: Pitsco Education-739068:3 ↔ Pitsco Education-739091:25
- Mate:268: Pitsco Education-739068:4 ↔ Pitsco Education-739066:1
- Flush:13: tetrix_739089_2012_MIR1:1 ↔ tetrix_739083_motor_2012_MIR1:1
- Mate:271: tetrix_739089_2012_MIR1:1 ↔ tetrix_739083_motor_2012_MIR1:1
- Mate:272: tetrix_739083_motor_2012_MIR1:1 ↔ tetrix_739079_2012_MIR:1
- Mate:273: tetrix_739083_motor_2012_MIR1:1 ↔ tetrix_739079_2012_MIR:1
- Mate:274: tetrix_739079_2012_MIR:1 ↔ tetrix_739165_sprk_25_16t_2013_MIR:1
- Mate:275: tetrix_739079_2012_MIR:1 ↔ tetrix_739165_sprk_25_16t_2013_MIR:1
- Mate:276: Pitsco Education-739068:1 ↔ tetrix_739089_2012_MIR1:1
- Mate:277: Pitsco Education-739068:1 ↔ tetrix_739089_2012_MIR1:1
- Flush:14: Pitsco Education-739068:1 ↔ Pitsco Education-739066:3
- Mate:278: Pitsco Education-739068:2 ↔ Pitsco Education-739066:3
- Mate:279: Pitsco Education-739066:3 ↔ tetrix_739089_2012_MIR1:1
- Mate:280: Pitsco Education-739066_MIR:1 ↔ tetrix_739089_2012_MIR1_MIR:1
- Mate:281: tetrix_739089_2012_MIR1_MIR:1 ↔ tetrix_739083_motor_2012_MIR1_MIR:1
- Flush:15: tetrix_739089_2012_MIR1_MIR:1 ↔ tetrix_739083_motor_2012_MIR1_MIR:1
- Mate:282: tetrix_739083_motor_2012_MIR1_MIR:1 ↔ tetrix_739079_2012_MIR_MIR:1
- Mate:283: tetrix_739083_motor_2012_MIR1_MIR:1 ↔ tetrix_739079_2012_MIR_MIR:1
- Mate:284: tetrix_739079_2012_MIR_MIR:1 ↔ tetrix_739165_sprk_25_16t_2013_MIR_MIR:1
- Mate:285: tetrix_739079_2012_MIR_MIR:1 ↔ tetrix_739165_sprk_25_16t_2013_MIR_MIR:1
- Flush:16: Pitsco Education-739068:1 ↔ Pitsco Education-739066_MIR:1
- Mate:286: Pitsco Education-739068:1 ↔ tetrix_739089_2012_MIR1_MIR:1
- Mate:287: Pitsco Education-739068:1 ↔ tetrix_739089_2012_MIR1_MIR:1
- Mate:288: Pitsco Education-739068:2 ↔ Pitsco Education-739066_MIR:1
- Mate:290: Pitsco Education-739068:3 ↔ Pitsco Education-739091:25
- Mate:291: Pitsco Education-739068:4 ↔ Pitsco Education-739091:24
- Mate:292: Pitsco Education-739091:25 ↔ Long Axle 250mm:2
- Mate:293: Pitsco Education-739068:3 ↔ Pitsco Education-739091:20
- Mate:294: Pitsco Education-739068:4 ↔ Pitsco Education-739091:21
- Mate:295 (254 mm): Pitsco Education-739068:4 ↔ Long Axle 250mm:1
- Mate:296: Pitsco Education-739091:21 ↔ Long Axle 250mm:1
- Mate:297 (254 mm): Pitsco Education-739068:4 ↔ Long Axle 250mm:2
- Mate:298: Long Axle 250mm:1 ↔ tetrix_739169_sprk_25_24t_2013:1
- Flush:17: tetrix_739165_sprk_25_16t_2013_MIR:1 ↔ tetrix_739169_sprk_25_24t_2013:1
- Mate:299: Long Axle 250mm:1 ↔ tetrix_739169_sprk_25_24t_2013:2
- Flush:18: tetrix_739165_sprk_25_16t_2013_MIR_MIR:1 ↔ tetrix_739169_sprk_25_24t_2013:2
- Mate:300: Long Axle 250mm:1 ↔ tetrix_739165_sprk_25_16t_2013:5
- Mate:301: Long Axle 250mm:1 ↔ tetrix_739165_sprk_25_16t_2013:7
- Mate:302 (25.4 mm): tetrix_739169_sprk_25_24t_2013:2 ↔ tetrix_739165_sprk_25_16t_2013:7
- Mate:303 (25.4 mm): tetrix_739169_sprk_25_24t_2013:1 ↔ tetrix_739165_sprk_25_16t_2013:5
- Mate:305: Long Axle 250mm:2 ↔ tetrix_739169_2012:2
- Flush:19: tetrix_739165_sprk_25_16t_2013:5 ↔ tetrix_739169_2012:2
- Flush:20: tetrix_739165_sprk_25_16t_2013:7 ↔ tetrix_739169_2012:1
- Mate:306: tetrix_739169_2012:1 ↔ tetrix_739172_collar_2012:10
- Mate:307: tetrix_739169_2012:1 ↔ tetrix_739172_collar_2012:10
- Mate:308: tetrix_739169_2012:2 ↔ tetrix_739172_collar_2012:9
- Mate:309: tetrix_739169_2012:2 ↔ tetrix_739172_collar_2012:9
- Mate:310: tetrix_739165_sprk_25_16t_2013:7 ↔ tetrix_739172_collar_2012:5
- Mate:311: tetrix_739165_sprk_25_16t_2013:7 ↔ tetrix_739172_collar_2012:5
- Mate:312: tetrix_739169_sprk_25_24t_2013:2 ↔ tetrix_739172_collar_2012:6
- Mate:313: tetrix_739169_sprk_25_24t_2013:2 ↔ tetrix_739172_collar_2012:6
- Mate:314: tetrix_739169_sprk_25_24t_2013:1 ↔ tetrix_739172_collar_2012:7
- Mate:315: tetrix_739169_sprk_25_24t_2013:1 ↔ tetrix_739172_collar_2012:7
- Mate:316: tetrix_739165_sprk_25_16t_2013:5 ↔ tetrix_739172_collar_2012:8
- Mate:317: tetrix_739165_sprk_25_16t_2013:5 ↔ tetrix_739172_collar_2012:8
- Mate:318: Long Axle 250mm:2 ↔ tetrix_739172_collar_2012:12
- Mate:320: Long Axle 250mm:2 ↔ tetrix_739068_2012:2
- Mate:321: tetrix_739068_2012:2 ↔ tetrix_739172_collar_2012:12
- Mate:323: Long Axle 250mm:2 ↔ tetrix_739068_2012:3
- Mate:324: Long Axle 250mm:2 ↔ tetrix_739172_collar_2012:13
- Mate:325: Pitsco Education-739068:4 ↔ tetrix_739068_2012:3
- Mate:326: tetrix_739068_2012:3 ↔ tetrix_739172_collar_2012:13
- Mate:328: Pitsco Education-739068:2 ↔ tetrix_991444_2012:3
- Mate:329: Pitsco Education-739068:2 ↔ tetrix_991444_2012:3
- Mate:330: Pitsco Education-739066:1 ↔ tetrix_991444_2012:5
- Mate:331: Pitsco Education-739068:4 ↔ tetrix_991444_2012:5
- Mate:332: Pitsco Education-739068:4 ↔ tetrix_991444_2012:5
- Mate:333: Pitsco Education-739066:2 ↔ tetrix_991444_2012:4
- Mate:334: Pitsco Education-739068:3 ↔ tetrix_991444_2012:4
- Flush:22: tetrix_991444_2012:4 ↔ tetrix_991444_2012:5
- Mate:335 (88.9 mm): Pitsco Education-739069:1 ↔ tetrix_739057_2012:1
- Flush:23: Pitsco Education-739069:1 ↔ tetrix_739057_2012:1
- Mate:336 (5.08 mm): Pitsco Education-739068:1 ↔ tetrix_739057_2012:1
- Mate:337: Long Axle 250mm:2 ↔ tetrix_739169_2012:1
- Mate:338: Pitsco Education-739068:3 ↔ Pitsco Education-739375:2
- Flush:24: Pitsco Education-739068:3 ↔ Pitsco Education-739375:2
- Mate:339: Pitsco Education-739068:3 ↔ Pitsco Education-739375:2
- Mate:340: Pitsco Education-739068:4 ↔ Pitsco Education-739375:1
- Flush:25: Pitsco Education-739068:4 ↔ Pitsco Education-739375:1
- Mate:341: Pitsco Education-739068:4 ↔ Pitsco Education-739375:1
- Mate:343: Pitsco Education-739068:3 ↔ tetrix_739068_2012:2
- Mate:344: tetrix_739068_2012:3 ↔ GAME ELEMENT FINAL:1
